# Autodesk Inventor assembly: 射出_モーター
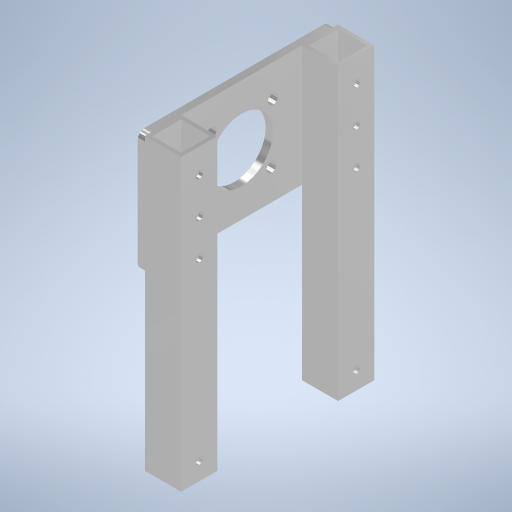
[picture p0: Inventor's stored thumbnail of the model, 512x512]
Saved by Autodesk Inventor 2023 (Build 270158000, 158)
## iProperties
Created: 2022-04-24
Part Number: 射出_モーター
Document SubType Name: Assembly
Designer: yuta
Author: yuta
## Documents named in this file (3)
- C:\Users\yuta\Documents\NHK\射出_モーター.iam
- C:\Users\yuta\Documents\NHK\射出_角柱1.ipt
- C:\Users\yuta\Documents\NHK\射出_モーター固定1.ipt
## Components (3 placed, 2 different names)
1. 射出_角柱1:2 — メイト:5, メイト:6, メイト:7, メイト:8
2. 射出_角柱1:3 — メイト:1, メイト:2, メイト:3, メイト:4
3. 射出_モーター固定1:1 — メイト:1, メイト:2, メイト:3, メイト:4, メイト:5, メイト:6, メイト:7, メイト:8
## Relationships (8: Mate 8)
- メイト:1 [Mate]: 射出_角柱1:3 ↔ 射出_モーター固定1:1
- メイト:2 [Mate]: 射出_角柱1:3 ↔ 射出_モーター固定1:1
- メイト:3 [Mate]: 射出_角柱1:3 ↔ 射出_モーター固定1:1
- メイト:4 [Mate]: 射出_角柱1:3 ↔ 射出_モーター固定1:1
- メイト:5 [Mate]: 射出_角柱1:2 ↔ 射出_モーター固定1:1
- メイト:6 [Mate]: 射出_角柱1:2 ↔ 射出_モーター固定1:1
- メイト:7 [Mate]: 射出_角柱1:2 ↔ 射出_モーター固定1:1
- メイト:8 [Mate]: 射出_角柱1:2 ↔ 射出_モーター固定1:1
